# Autodesk Inventor assembly: 0603
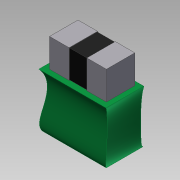
[picture p0: Inventor's stored thumbnail of the model, 180x180]
Saved by Autodesk Inventor 2011 (Build 150239000, 239)
## iProperties
Created: 2010-12-28
Part Number: 0603
Document SubType Name: Assembly
Designer: abbath
Author: abbath
## Documents named in this file (3)
- D:\Abbath\Work\11.2\Сумматор light\КД\RSXX к сумматору\Установка элементов\0603 установка.iam
- D:\Abbath\Work\11.2\Сумматор light\КД\RSXX к сумматору\Установка элементов\0603.ipt
- D:\Abbath\Work\11.2\Сумматор light\КД\RSXX к сумматору\Установка элементов\0603 плата.ipt
## Components (2 placed, 2 different names)
1. 0603:1 — Заподлицо:1
2. 0603 плата:1 — Заподлицо:1
## Relationships (1: Flush 1)
- Заподлицо:1 [Flush]: 0603:1 ↔ 0603 плата:1
